# Autodesk Inventor assembly: assembly
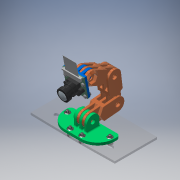
[picture p0: Inventor's stored thumbnail of the model, 180x180]
Saved by Autodesk Inventor 2018 (Build 220112000, 112)
## iProperties
Created: 2019-10-09
Part Number: assembly
Document SubType Name: Assembly
Designer: ZEUSLAP
Author: ZEUSLAP
## Documents named in this file (10)
- C:\data\Tonic\cad\camera_mount\assembly.iam
- C:\data\Tonic\cad\camera_mount\parts\platform.ipt
- C:\data\Tonic\cad\camera_mount\printable\camera_mount.ipt
- C:\data\Tonic\cad\camera_mount\printable\platform_mount.ipt
- C:\data\Tonic\cad\camera_mount\parts\camera\Raspberry Pi Camera (G) 160 deg.iam
- C:\data\Tonic\cad\camera_mount\printable\arm-30-straight-v5-1.ipt
- C:\Users\ZEUSLAP\Documents\Inventor\Content Center Files\R2018\en-US\ISO 4035(2)\ISO 4035 - M3 - ISO.ipt
- C:\Users\ZEUSLAP\Documents\Inventor\Content Center Files\R2018\en-US\SFS EN ISO 7045 Z\EN ISO 7045 - M3 x 8 - 4.8 - Z(3).ipt
- C:\Users\ZEUSLAP\Documents\Inventor\Content Center Files\R2018\en-US\SFS EN ISO 7045 Z\EN ISO 7045 - M2 x 5 - 4.8 - Z(3).ipt
- C:\Users\ZEUSLAP\Documents\Inventor\Content Center Files\R2018\en-US\ISO 4035(2)\ISO 4035 - M2 - ISO.ipt
## Components (23 placed, 9 different names)
1. platform:1 — Mate:1, Mate:2, Mate:3, Mate:46, Mate:47, Mate:48, Mate:49, Mate:50, Mate:51, Mate:52, Mate:53
2. camera_mount:1 — Mate:10, Mate:11, Mate:12, Mate:13, Mate:39, Mate:41, Mate:43, Mate:45
3. platform_mount:1 — Mate:1, Mate:2, Mate:3, Mate:4, Mate:5, Mate:55, Mate:57, Mate:59, Mate:61, Angle:1, Angle:2, Angle:3, Angle:4
4. Raspberry Pi Camera (G) 160 deg:1 [sub-assembly] — Mate:12, Mate:13, Mate:30, Mate:31, Mate:32, Mate:33, Mate:34, Mate:35, Mate:36, Mate:37
5. arm-30-straight-v5-1:1 — Mate:8, Mate:9, Mate:10, Mate:11
6. arm-30-straight-v5-1:2 — Mate:4, Mate:5, Mate:6, Mate:7
7. arm-30-straight-v5-1:3 — Mate:6, Mate:7, Mate:8, Mate:9
8. SFS EN ISO 7045 Z M2 x 5 - 4.8 - Z:1 — Mate:30, Mate:31, Mate:38
9. SFS EN ISO 7045 Z M2 x 5 - 4.8 - Z:2 — Mate:32, Mate:33, Mate:42
10. SFS EN ISO 7045 Z M2 x 5 - 4.8 - Z:3 — Mate:34, Mate:35, Mate:44
11. SFS EN ISO 7045 Z M2 x 5 - 4.8 - Z:4 — Mate:36, Mate:37, Mate:40
12. ISO 4035 M2:1 — Mate:38, Mate:39
13. ISO 4035 M2:2 — Mate:40, Mate:41
14. ISO 4035 M2:3 — Mate:42, Mate:43
15. ISO 4035 M2:4 — Mate:44, Mate:45
16. SFS EN ISO 7045 Z M3 x 8 - 4.8 - Z:1 — Mate:46, Mate:47, Mate:56
17. SFS EN ISO 7045 Z M3 x 8 - 4.8 - Z:2 — Mate:48, Mate:49, Mate:58
18. SFS EN ISO 7045 Z M3 x 8 - 4.8 - Z:3 — Mate:50, Mate:51, Mate:54
19. SFS EN ISO 7045 Z M3 x 8 - 4.8 - Z:4 — Mate:52, Mate:53, Mate:60
20. ISO 4035 M3:1 — Mate:54, Mate:55, Angle:2
21. ISO 4035 M3:2 — Mate:56, Mate:57, Angle:3
22. ISO 4035 M3:3 — Mate:58, Mate:59, Angle:4
23. ISO 4035 M3:4 — Mate:60, Mate:61, Angle:1
## Relationships (49: Mate 45, Angle 4)
- Mate:1: platform:1 ↔ platform_mount:1
- Mate:2: platform:1 ↔ platform_mount:1
- Mate:3: platform:1 ↔ platform_mount:1
- Mate:4: platform_mount:1 ↔ arm-30-straight-v5-1:2
- Mate:5: platform_mount:1 ↔ arm-30-straight-v5-1:2
- Mate:6: arm-30-straight-v5-1:2 ↔ arm-30-straight-v5-1:3
- Mate:7: arm-30-straight-v5-1:2 ↔ arm-30-straight-v5-1:3
- Mate:8: arm-30-straight-v5-1:1 ↔ arm-30-straight-v5-1:3
- Mate:9: arm-30-straight-v5-1:1 ↔ arm-30-straight-v5-1:3
- Mate:10: camera_mount:1 ↔ arm-30-straight-v5-1:1
- Mate:11: camera_mount:1 ↔ arm-30-straight-v5-1:1
- Mate:12: camera_mount:1 ↔ Raspberry Pi Camera (G) 160 deg:1
- Mate:13: camera_mount:1 ↔ Raspberry Pi Camera (G) 160 deg:1
- Mate:30: Raspberry Pi Camera (G) 160 deg:1 ↔ SFS EN ISO 7045 Z M2 x 5 - 4.8 - Z:1
- Mate:31: Raspberry Pi Camera (G) 160 deg:1 ↔ SFS EN ISO 7045 Z M2 x 5 - 4.8 - Z:1
- Mate:32: Raspberry Pi Camera (G) 160 deg:1 ↔ SFS EN ISO 7045 Z M2 x 5 - 4.8 - Z:2
- Mate:33: Raspberry Pi Camera (G) 160 deg:1 ↔ SFS EN ISO 7045 Z M2 x 5 - 4.8 - Z:2
- Mate:34: Raspberry Pi Camera (G) 160 deg:1 ↔ SFS EN ISO 7045 Z M2 x 5 - 4.8 - Z:3
- Mate:35: Raspberry Pi Camera (G) 160 deg:1 ↔ SFS EN ISO 7045 Z M2 x 5 - 4.8 - Z:3
- Mate:36: Raspberry Pi Camera (G) 160 deg:1 ↔ SFS EN ISO 7045 Z M2 x 5 - 4.8 - Z:4
- Mate:37: Raspberry Pi Camera (G) 160 deg:1 ↔ SFS EN ISO 7045 Z M2 x 5 - 4.8 - Z:4
- Mate:38: SFS EN ISO 7045 Z M2 x 5 - 4.8 - Z:1 ↔ ISO 4035 M2:1
- Mate:39: camera_mount:1 ↔ ISO 4035 M2:1
- Mate:40: SFS EN ISO 7045 Z M2 x 5 - 4.8 - Z:4 ↔ ISO 4035 M2:2
- Mate:41: camera_mount:1 ↔ ISO 4035 M2:2
- Mate:42: SFS EN ISO 7045 Z M2 x 5 - 4.8 - Z:2 ↔ ISO 4035 M2:3
- Mate:43: camera_mount:1 ↔ ISO 4035 M2:3
- Mate:44: SFS EN ISO 7045 Z M2 x 5 - 4.8 - Z:3 ↔ ISO 4035 M2:4
- Mate:45: camera_mount:1 ↔ ISO 4035 M2:4
- Mate:46: platform:1 ↔ SFS EN ISO 7045 Z M3 x 8 - 4.8 - Z:1
- Mate:47: platform:1 ↔ SFS EN ISO 7045 Z M3 x 8 - 4.8 - Z:1
- Mate:48: platform:1 ↔ SFS EN ISO 7045 Z M3 x 8 - 4.8 - Z:2
- Mate:49: platform:1 ↔ SFS EN ISO 7045 Z M3 x 8 - 4.8 - Z:2
- Mate:50: platform:1 ↔ SFS EN ISO 7045 Z M3 x 8 - 4.8 - Z:3
- Mate:51: platform:1 ↔ SFS EN ISO 7045 Z M3 x 8 - 4.8 - Z:3
- Mate:52: platform:1 ↔ SFS EN ISO 7045 Z M3 x 8 - 4.8 - Z:4
- Mate:53: platform:1 ↔ SFS EN ISO 7045 Z M3 x 8 - 4.8 - Z:4
- Mate:54: SFS EN ISO 7045 Z M3 x 8 - 4.8 - Z:3 ↔ ISO 4035 M3:1
- Mate:55: platform_mount:1 ↔ ISO 4035 M3:1
- Mate:56: SFS EN ISO 7045 Z M3 x 8 - 4.8 - Z:1 ↔ ISO 4035 M3:2
- Mate:57: platform_mount:1 ↔ ISO 4035 M3:2
- Mate:58: SFS EN ISO 7045 Z M3 x 8 - 4.8 - Z:2 ↔ ISO 4035 M3:3
- Mate:59: platform_mount:1 ↔ ISO 4035 M3:3
- Mate:60: SFS EN ISO 7045 Z M3 x 8 - 4.8 - Z:4 ↔ ISO 4035 M3:4
- Mate:61: platform_mount:1 ↔ ISO 4035 M3:4
- Angle:1 (90 deg): platform_mount:1 ↔ ISO 4035 M3:4
- Angle:2 (90 deg): platform_mount:1 ↔ ISO 4035 M3:1
- Angle:3 (90 deg): platform_mount:1 ↔ ISO 4035 M3:2
- Angle:4 (90 deg): platform_mount:1 ↔ ISO 4035 M3:3
